# Autodesk Inventor assembly: Linear Actuator
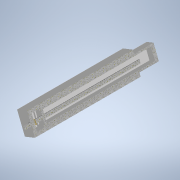
[picture p0: Inventor's stored thumbnail of the model, 180x180]
Saved by Autodesk Inventor 2021 (Build 250183000, 183)
## iProperties
Created: 2021-08-04
Part Number: Linear Actuator
Document SubType Name: Assembly
Designer: techv
Author: techv
## Documents named in this file (4)
- D:\Projects\P_Borewell\V2\Design of piston cylinder\Linear Actuator.iam
- D:\Projects\P_Borewell\V2\Design of piston cylinder\Lead Screw.ipt
- D:\Projects\P_Borewell\V2\Design of piston cylinder\Nut.ipt
- D:\Projects\P_Borewell\V2\Design of piston cylinder\Casing.ipt
## Components (3 placed, 3 different names)
1. Lead Screw:1 — Mate:1, Flush:1
2. Piston — Mate:1, Mate:2, Mate:3, Mate:4, Flush:2
3. Casing:1 — Flush:1, Mate:2, Mate:3, Mate:4, Flush:2
## Relationships (6: Mate 4, Flush 2)
- Mate:1: Lead Screw:1 ↔ Piston
- Flush:1 (-5 mm): Lead Screw:1 ↔ Casing:1
- Mate:2: Piston ↔ Casing:1
- Mate:3: Piston ↔ Casing:1
- Mate:4: Piston ↔ Casing:1
- Flush:2: Piston ↔ Casing:1
